# Autodesk Inventor assembly: GE-18032
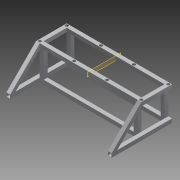
[picture p0: Inventor's stored thumbnail of the model, 180x180]
Saved by Autodesk Inventor 2018 (Build 220112000, 112)
## iProperties
Created: 2017-12-19
Part Number: GE-18032
Document SubType Name: Assembly
Designer: PhillipD
Author: PhillipD
Revision Number: ANY
## Documents named in this file (7)
- D:\FIRST 2018\FIRST 2018 Inventor\FIRST 2018 Field\Parts\GE-18032.iam
- D:\FIRST 2018\FIRST 2018 Inventor\FIRST 2018 Field\Parts\GE-18032-01.ipt
- D:\FIRST 2018\FIRST 2018 Inventor\FIRST 2018 Field\Parts\GE-18032-02.ipt
- D:\FIRST 2018\FIRST 2018 Inventor\FIRST 2018 Field\Parts\GE-18032-03.ipt
- D:\FIRST 2018\FIRST 2018 Inventor\FIRST 2018 Field\Parts\GE-18032-05.ipt
- D:\FIRST 2018\FIRST 2018 Inventor\FIRST 2018 Field\Parts\GE-18032-04.ipt
- D:\FIRST 2018\FIRST 2018 Inventor\FIRST 2018 Field\Parts\GE-18032-06.ipt
## Components (14 placed, 14 different names)
1. GE-18032-01_174
2. GE-18032-02_175 — Symmetry:1, Symmetry:2
3. GE-18032-03_176
4. GE-18032-05_177
5. GE-18032-04_178
6. GE-18032-06_179
7. GE-18032-01_180
8. GE-18032-02_181 — Symmetry:1, Symmetry:2
9. GE-18032-05_182
10. GE-18032-03_183
11. GE-18032-03_184
12. GE-18032-03_185
13. GE-18032-04_186
14. GE-18032-06_187
## Relationships (2: Symmetry 2)
- Symmetry:1: GE-18032-02_175 ↔ GE-18032-02_181
- Symmetry:2: GE-18032-02_175 ↔ GE-18032-02_181
